# Autodesk Inventor assembly: wheel1_MIR2
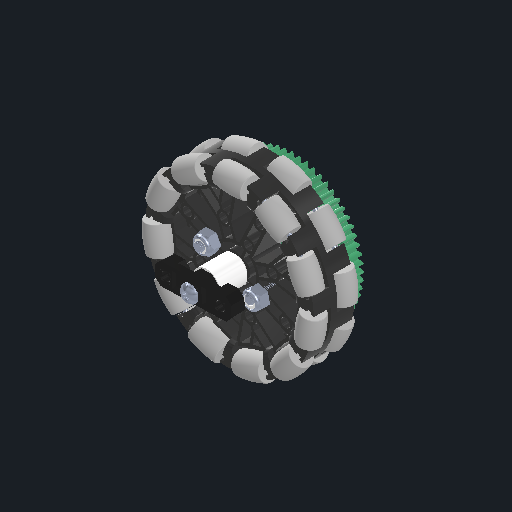
[picture p0: Inventor's stored thumbnail of the model, 512x512]
Saved by Autodesk Inventor 2024 (Build 280153000, 153)
## iProperties
Created: 2023-08-09
Part Number: wheel1_MIR2
Document SubType Name: Assembly
Designer: macbook
Author: macbook
## Documents named in this file (16)
- \\Mac\Home\Desktop\code\7899V-VRC-OVER-UNDER\Cad\VEX-CAD-Inventor-1.4.0\Assembly\v0.2\wheel1_MIR2.iam
- \\Mac\Home\Desktop\code\7899V-VRC-OVER-UNDER\Cad\VEX-CAD-Inventor-1.4.0\Motion\Wheels\Omni Wheel\3.25 Omni AS, Circle_MIR2.iam
- \\Mac\Home\Desktop\code\7899V-VRC-OVER-UNDER\Cad\VEX-CAD-Inventor-1.4.0\Motion\Spacers\Washer Teflon\TWasher .375 OD x .03125.ipt
- \\Mac\Home\Desktop\code\7899V-VRC-OVER-UNDER\Cad\VEX-CAD-Inventor-1.4.0\Motion\Spacers\Washer Teflon.ipt
- \\Mac\Home\Desktop\code\7899V-VRC-OVER-UNDER\Cad\VEX-CAD-Inventor-1.4.0\Motion\Shaft LS\Bearing Flat_MIR3.ipt
- \\Mac\Home\Desktop\code\7899V-VRC-OVER-UNDER\Cad\VEX-CAD-Inventor-1.4.0\Motion\Gears\LS 60T Gear_MIR1.ipt
- \\Mac\Home\Desktop\code\7899V-VRC-OVER-UNDER\Cad\VEX-CAD-Inventor-1.4.0\Structure\Hardware\Screw Steel - Star\SScrew Star Threaded 1.250.ipt
- \\Mac\Home\Desktop\code\7899V-VRC-OVER-UNDER\Cad\VEX-CAD-Inventor-1.4.0\Structure\Hardware\Screw Steel - Star.ipt
- \\Mac\Home\Desktop\code\7899V-VRC-OVER-UNDER\Cad\VEX-CAD-Inventor-1.4.0\Structure\Hardware\Nut Nylock_MIR3.ipt
- \\Mac\Home\Desktop\code\7899V-VRC-OVER-UNDER\Cad\VEX-CAD-Inventor-1.4.0\Structure\Hardware\Screw Steel - Star\SScrew Star Smooth 2.500.ipt
- \\Mac\Home\Desktop\code\7899V-VRC-OVER-UNDER\Cad\VEX-CAD-Inventor-1.4.0\Structure\C Channel\Aluminum 1x2x1\Alu C 1x2x1x14_MIR.ipt
- \\Mac\Home\Desktop\code\7899V-VRC-OVER-UNDER\Cad\VEX-CAD-Inventor-1.4.0\Motion\Spacers\Spacer Nylon .500 OD\NSpacer White .500 OD x .500.ipt
- \\Mac\Home\Desktop\code\7899V-VRC-OVER-UNDER\Cad\VEX-CAD-Inventor-1.4.0\Motion\Spacers\Spacer Nylon .500 OD.ipt
- \\Mac\Home\Desktop\code\7899V-VRC-OVER-UNDER\Cad\VEX-CAD-Inventor-1.4.0\Motion\Spacers\Washer Steel\SWasher .375 OD x .015625.ipt
- \\Mac\Home\Desktop\code\7899V-VRC-OVER-UNDER\Cad\VEX-CAD-Inventor-1.4.0\Motion\Spacers\Washer Steel.ipt
- \\Mac\Home\Desktop\code\7899V-VRC-OVER-UNDER\Cad\VEX-CAD-Inventor-1.4.0\Motion\Spacers\Spacer Nylon .500 OD\NSpacer White .500 OD x .375.ipt
## Components (19 placed, 11 different names)
1. 3.25 Omni AS, Circle_MIR2:1 [sub-assembly] — Insert:55, Insert:56, Insert:89, Insert:92
2. TWasher .375 OD x .03125:1 — Insert:68, Insert:36
3. Bearing Flat_MIR3:1 — Insert:47, Insert:46, Insert:71, Insert:36
4. Bearing Flat_MIR3:2 — Insert:47, Insert:46, Insert:70, Insert:73, Insert:72
5. LS 60T Gear_MIR1:1 — Insert:68, Insert:82, Insert:84, Insert:86, Insert:91
6. SScrew Star Threaded 1.250:1 — Insert:83
7. Nut Nylock_MIR3:1 — Insert:55
8. Nut Nylock_MIR3:2 — Insert:56
9. SScrew Star Threaded 1.250:2 — Insert:85
10. SScrew Star Smooth 2.500:3 — Insert:70
11. Nut Nylock_MIR3:3 — Insert:71
12. Alu C 1x2x1x14_MIR:1 — Insert:73, Insert:72
13. NSpacer White .500 OD x .500:1 — Insert:89, Insert:93
14. SWasher .375 OD x .015625:1 — Insert:82, Insert:81
15. NSpacer White .500 OD x .375:2 — Insert:81
16. TWasher .375 OD x .03125:2 — Insert:84, Insert:83
17. TWasher .375 OD x .03125:3 — Insert:86, Insert:85
18. TWasher .375 OD x .03125:4 — Insert:93
19. NSpacer White .500 OD x .375:3 — Insert:92, Insert:91
## Relationships (20: Insert 20)
- Insert:47 (44.45 mm): Bearing Flat_MIR3:1 ↔ Bearing Flat_MIR3:2
- Insert:46 (44.45 mm): Bearing Flat_MIR3:1 ↔ Bearing Flat_MIR3:2
- Insert:55: 3.25 Omni AS, Circle_MIR2:1 ↔ Nut Nylock_MIR3:1
- Insert:56: 3.25 Omni AS, Circle_MIR2:1 ↔ Nut Nylock_MIR3:2
- Insert:70 (1.5875 mm): Bearing Flat_MIR3:2 ↔ SScrew Star Smooth 2.500:3
- Insert:71: Bearing Flat_MIR3:1 ↔ Nut Nylock_MIR3:3
- Insert:73: Bearing Flat_MIR3:2 ↔ Alu C 1x2x1x14_MIR:1
- Insert:72: Bearing Flat_MIR3:2 ↔ Alu C 1x2x1x14_MIR:1
- Insert:89: 3.25 Omni AS, Circle_MIR2:1 ↔ NSpacer White .500 OD x .500:1
- Insert:68: TWasher .375 OD x .03125:1 ↔ LS 60T Gear_MIR1:1
- Insert:36 (1.5875 mm): TWasher .375 OD x .03125:1 ↔ Bearing Flat_MIR3:1
- Insert:82: LS 60T Gear_MIR1:1 ↔ SWasher .375 OD x .015625:1
- Insert:81: SWasher .375 OD x .015625:1 ↔ NSpacer White .500 OD x .375:2
- Insert:84: LS 60T Gear_MIR1:1 ↔ TWasher .375 OD x .03125:2
- Insert:83: SScrew Star Threaded 1.250:1 ↔ TWasher .375 OD x .03125:2
- Insert:86: LS 60T Gear_MIR1:1 ↔ TWasher .375 OD x .03125:3
- Insert:85: SScrew Star Threaded 1.250:2 ↔ TWasher .375 OD x .03125:3
- Insert:93: NSpacer White .500 OD x .500:1 ↔ TWasher .375 OD x .03125:4
- Insert:92: 3.25 Omni AS, Circle_MIR2:1 ↔ NSpacer White .500 OD x .375:3
- Insert:91: LS 60T Gear_MIR1:1 ↔ NSpacer White .500 OD x .375:3
